# Autodesk Inventor assembly: 276-2162
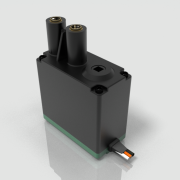
[picture p0: Inventor's stored thumbnail of the model, 180x180]
Saved by Autodesk Inventor 2015 SP1 (Build 190201100, 201)
## iProperties
Category: Motion
Company: Super Sonic Sparks, Team 24
Part Number: 276-2162
Document SubType Name: Assembly
Designer: Jordan Kiesel
Mass: 43.545 g
Surface Area: 235.545 cm^2
Volume: 14.3379 cm^3
Density: 3.03706 g/cm^3
Catalog Web Link: vexrobotics.com/276-2162.html
Description: Can be directed to turn to face a speciﬁc direction.
Vendor: VEX Robotics, Inc.
Translation Standard: STEP AP203
FileName: 3-Wire Servo Motor.iam
PreProcessor: SolidWorks 2006052
PostProcessor: Build: 239, Release: 2011 RTM - Date: Wed 02/17/2010
Sent Units: inch
Uncertainty: 1e-05
Author: Jordan Kiesel
Title: 3-Wire Servo Motor
Comments: Servo motors are a type of motor that can be directed to turn to face a speciﬁc direction, rather than just spin forward or backward. ▷ Expand functionality ▷ Add pan and tilt to a camera ▷ 100 degrees of rotation ▷ Do exact positioning
## Documents named in this file (12)
- C:\Users\Jordan\Documents\Robotics\VEX\CAD\2015 BNS CAD Library (beta)\Motion\Motors\3-Wire Servo Motor.iam
- C:\Users\Jordan\Documents\Robotics\VEX\CAD\2015 BNS CAD Library (beta)\Motion\Motors\Reference Parts\3-Wire Motors\6-32 Screw Insert Nut.ipt
- C:\Users\Jordan\Documents\Robotics\VEX\CAD\2015 BNS CAD Library (beta)\Motion\Motors\Reference Parts\3-Wire Motors\Top Housing.ipt
- C:\Users\Jordan\Documents\Robotics\VEX\CAD\2015 BNS CAD Library (beta)\Motion\Motors\Reference Parts\3-Wire Motors\Bottom Housing.ipt
- C:\Users\Jordan\Documents\Robotics\VEX\CAD\2015 BNS CAD Library (beta)\Motion\Motors\Reference Parts\Motors\3-Wire Cable Support.ipt
- C:\Users\Jordan\Documents\Robotics\VEX\CAD\2015 BNS CAD Library (beta)\Motion\Motors\Reference Parts\Motors\3-Wire Black-Orange-White Cable, Cut.ipt
- C:\Users\Jordan\Documents\Robotics\VEX\CAD\2015 BNS CAD Library (beta)\Motion\Motors\Reference Parts\3-Wire Motors\Screw.ipt
- C:\Users\Jordan\Documents\Robotics\VEX\CAD\2015 BNS CAD Library (beta)\Motion\Motors\Reference Parts\3-Wire Motors\33-tooth Output Gear.ipt
- C:\Users\Jordan\Documents\Robotics\VEX\CAD\2015 BNS CAD Library (beta)\Motion\Motors\Reference Parts\3-Wire Motors\Bottom Plate.ipt
- C:\Users\Jordan\Documents\Robotics\VEX\CAD\2015 BNS CAD Library (beta)\Motion\Motors\Reference Parts\3-Wire Motors\11-40-tooth Compound Gear.ipt
- C:\Users\Jordan\Documents\Robotics\VEX\CAD\2015 BNS CAD Library (beta)\Motion\Motors\Reference Parts\3-Wire Motors\12-50-tooth Compound Gear.ipt
- C:\Users\Jordan\Documents\Robotics\VEX\CAD\2015 BNS CAD Library (beta)\Motion\Motors\Reference Parts\3-Wire Motors\14-50-tooth Compound Gear.ipt
## Components (19 placed, 11 different names)
1. Screw:1 — Insert:12
2. 6-32 Screw Insert Nut:1 — Insert:8
3. Top Housing:1 — Insert:7, Insert:8, Insert:9, Insert:10, Insert:11, Insert:12, Insert:13, Insert:14, Insert:15, Insert:16
4. Screw:2 — Insert:3
5. 33-tooth Output Gear:1 — Insert:15, Rotation:1, Angle:1
6. 6-32 Screw Insert Nut:2 — Insert:7
7. Screw:3 — Insert:9
8. Bottom Plate:1 — Insert:1, Insert:2, Insert:3, Insert:4, Insert:5, Insert:6
9. Screw:4 — Insert:11
10. Bottom Housing:1 — Insert:5, Insert:6, Insert:13, Insert:14, Insert:17, Insert:18
11. Screw:5 — Insert:1
12. Screw:6 — Insert:10
13. 3-Wire Cable Support:1 — Angle:1
14. Screw:7 — Insert:2
15. Screw:8 — Insert:4
16. 3-Wire Black-Orange-White Cable, Cut:1
17. 11-40-tooth Compound Gear:1 — Insert:16, Rotation:1, Rotation:2
18. 12-50-tooth Compound Gear:1 — Insert:17, Rotation:2, Rotation:3
19. 14-50-tooth Compound Gear:1 — Insert:18, Rotation:3
## Relationships (22: Insert 18, RelateRotation 3, Angle 1)
- Insert:1: Bottom Plate:1 ↔ Screw:5
- Insert:2: Bottom Plate:1 ↔ Screw:7
- Insert:3: Screw:2 ↔ Bottom Plate:1
- Insert:4: Bottom Plate:1 ↔ Screw:8
- Insert:5: Bottom Plate:1 ↔ Bottom Housing:1
- Insert:6: Bottom Plate:1 ↔ Bottom Housing:1
- Insert:7 (0.127 mm): Top Housing:1 ↔ 6-32 Screw Insert Nut:2
- Insert:8 (0.127 mm): 6-32 Screw Insert Nut:1 ↔ Top Housing:1
- Insert:9: Top Housing:1 ↔ Screw:3
- Insert:10: Top Housing:1 ↔ Screw:6
- Insert:11: Top Housing:1 ↔ Screw:4
- Insert:12: Screw:1 ↔ Top Housing:1
- Insert:13: Top Housing:1 ↔ Bottom Housing:1
- Insert:14: Top Housing:1 ↔ Bottom Housing:1
- Insert:15: Top Housing:1 ↔ 33-tooth Output Gear:1
- Insert:16: Top Housing:1 ↔ 11-40-tooth Compound Gear:1
- Insert:17: Bottom Housing:1 ↔ 12-50-tooth Compound Gear:1
- Insert:18: Bottom Housing:1 ↔ 14-50-tooth Compound Gear:1
- Rotation:1 [RelateRotation] (3 ul): 33-tooth Output Gear:1 ↔ 11-40-tooth Compound Gear:1
- Rotation:2 [RelateRotation] (3.3333 ul): 11-40-tooth Compound Gear:1 ↔ 12-50-tooth Compound Gear:1
- Rotation:3 [RelateRotation] (3.5714 ul): 12-50-tooth Compound Gear:1 ↔ 14-50-tooth Compound Gear:1
- Angle:1 (0 deg): 33-tooth Output Gear:1 ↔ 3-Wire Cable Support:1
